# Autodesk Inventor assembly: GP2-100
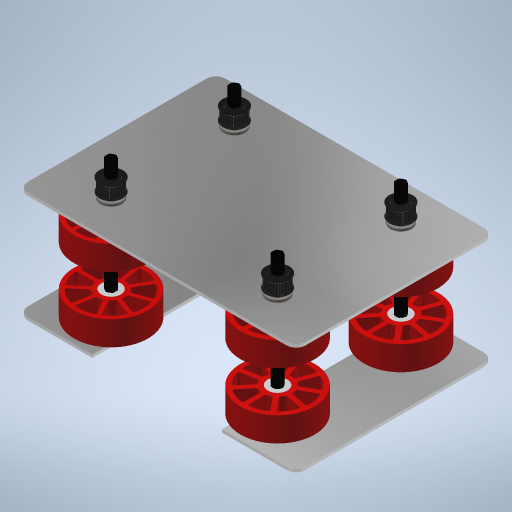
[picture p0: Inventor's stored thumbnail of the model, 512x512]
Saved by Autodesk Inventor 2023.4 (Build 274418000, 418)
## iProperties
Created: 2025-01-12
Part Number: GP2-100
Document SubType Name: Assembly
Designer: jmcintyr
Author: jmcintyr
## Documents named in this file (8)
- C:\Users\jmcintyr\Desktop\2025-ReefScape---CAD\Gripper\GP2\GP2-100.iam
- C:\Users\jmcintyr\Desktop\2025-ReefScape---CAD\Gripper\GP2\GP2-002.ipt
- C:\Users\jmcintyr\Desktop\2025-ReefScape---CAD\Gripper\GP2\GP2-001.ipt
- C:\Users\jmcintyr\Desktop\2025-ReefScape---CAD\COMMON PARTS\BEARINGS\10_25mm_3_8_ThunderHex_ID_x_0_875_OD_x_0_280_WD_Flanged_Bearing_217-5829.ipt
- C:\Users\jmcintyr\Desktop\2025-ReefScape---CAD\Gripper\GP2\GP2-002_MIR4.ipt
- C:\Users\jmcintyr\Desktop\2025-ReefScape---CAD\COMMON PARTS\WHEELS\am-3946 3IN 375Hex Compliant Wheel REV 3.ipt
- C:\Users\jmcintyr\Desktop\2025-ReefScape---CAD\Gripper\GP2\.375_ThunderHex.ipt
- C:\Users\jmcintyr\Desktop\2025-ReefScape---CAD\COMMON PARTS\PULLEYS\gt2\24T_GT2_375_HexBore_9mm_wide_Flanged_Pulley.ipt
## Components (27 placed, 7 different names)
1. GP2-002:1 — Flush:1, Flush:2, Flush:3, Flush:8, Insert:1, Insert:2, Insert:3
2. GP2-001:1 — Flush:8, Insert:1, Insert:4, Insert:5, Insert:8, Insert:9
3. 10_25mm_3_8_ThunderHex_ID_x_0_875_OD_x_0_280_WD_Flanged_Bearing_217-5829:1 — Insert:9, Insert:16, Insert:26
4. 10_25mm_3_8_ThunderHex_ID_x_0_875_OD_x_0_280_WD_Flanged_Bearing_217-5829:2 — Insert:8, Insert:17, Insert:27
5. 10_25mm_3_8_ThunderHex_ID_x_0_875_OD_x_0_280_WD_Flanged_Bearing_217-5829:3 — Insert:5, Insert:14, Insert:25
6. 10_25mm_3_8_ThunderHex_ID_x_0_875_OD_x_0_280_WD_Flanged_Bearing_217-5829:4 — Insert:4, Insert:15, Insert:24
7. 10_25mm_3_8_ThunderHex_ID_x_0_875_OD_x_0_280_WD_Flanged_Bearing_217-5829:5 — Insert:10, Insert:19, Insert:20
8. 10_25mm_3_8_ThunderHex_ID_x_0_875_OD_x_0_280_WD_Flanged_Bearing_217-5829:6 — Insert:11, Insert:18, Insert:23
9. 10_25mm_3_8_ThunderHex_ID_x_0_875_OD_x_0_280_WD_Flanged_Bearing_217-5829:7 — Insert:2, Insert:12, Insert:21
10. 10_25mm_3_8_ThunderHex_ID_x_0_875_OD_x_0_280_WD_Flanged_Bearing_217-5829:8 — Insert:3, Insert:13, Insert:22
11. GP2-002_MIR4:1 — Flush:9, Flush:10, Flush:11, Insert:10, Insert:11
12. am-3946 3IN 375Hex Compliant Wheel REV 3:1 — Insert:15
13. am-3946 3IN 375Hex Compliant Wheel REV 3:2 — Insert:14
14. am-3946 3IN 375Hex Compliant Wheel REV 3:3 — Insert:13
15. am-3946 3IN 375Hex Compliant Wheel REV 3:4 — Insert:12
16. am-3946 3IN 375Hex Compliant Wheel REV 3:5 — Insert:18
17. am-3946 3IN 375Hex Compliant Wheel REV 3:6 — Insert:17
18. am-3946 3IN 375Hex Compliant Wheel REV 3:7 — Insert:16
19. am-3946 3IN 375Hex Compliant Wheel REV 3:8 — Insert:19
20. .375_ThunderHex:1 — Insert:20
21. .375_ThunderHex:2 — Insert:23
22. .375_ThunderHex:3 — Insert:22
23. .375_ThunderHex:4 — Insert:21
24. 24T_GT2_375_HexBore_9mm_wide_Flanged_Pulley:1 — Insert:27
25. 24T_GT2_375_HexBore_9mm_wide_Flanged_Pulley:2 — Insert:24
26. 24T_GT2_375_HexBore_9mm_wide_Flanged_Pulley:3 — Insert:25
27. 24T_GT2_375_HexBore_9mm_wide_Flanged_Pulley:4 — Insert:26
## Relationships (35: Insert 25, Flush 7, Mate 2, Angle 1)
- Mate:1
- Angle:1 (0 deg)
- Flush:1 (-19.05 mm): GP2-002:1
- Mate:2 (85.725 mm)
- Flush:2: GP2-002:1
- Flush:3: GP2-002:1
- Flush:8: GP2-002:1 ↔ GP2-001:1
- Insert:1 (107.95 mm): GP2-002:1 ↔ GP2-001:1
- Insert:2: GP2-002:1 ↔ 10_25mm_3_8_ThunderHex_ID_x_0_875_OD_x_0_280_WD_Flanged_Bearing_217-5829:7
- Insert:3: GP2-002:1 ↔ 10_25mm_3_8_ThunderHex_ID_x_0_875_OD_x_0_280_WD_Flanged_Bearing_217-5829:8
- Insert:4: GP2-001:1 ↔ 10_25mm_3_8_ThunderHex_ID_x_0_875_OD_x_0_280_WD_Flanged_Bearing_217-5829:4
- Insert:5: GP2-001:1 ↔ 10_25mm_3_8_ThunderHex_ID_x_0_875_OD_x_0_280_WD_Flanged_Bearing_217-5829:3
- Insert:8: GP2-001:1 ↔ 10_25mm_3_8_ThunderHex_ID_x_0_875_OD_x_0_280_WD_Flanged_Bearing_217-5829:2
- Insert:9: GP2-001:1 ↔ 10_25mm_3_8_ThunderHex_ID_x_0_875_OD_x_0_280_WD_Flanged_Bearing_217-5829:1
- Flush:9: GP2-002_MIR4:1
- Flush:10: GP2-002_MIR4:1
- Flush:11 (-19.05 mm): GP2-002_MIR4:1
- Insert:10: 10_25mm_3_8_ThunderHex_ID_x_0_875_OD_x_0_280_WD_Flanged_Bearing_217-5829:5 ↔ GP2-002_MIR4:1
- Insert:11: 10_25mm_3_8_ThunderHex_ID_x_0_875_OD_x_0_280_WD_Flanged_Bearing_217-5829:6 ↔ GP2-002_MIR4:1
- Insert:12 (3.175 mm): 10_25mm_3_8_ThunderHex_ID_x_0_875_OD_x_0_280_WD_Flanged_Bearing_217-5829:7 ↔ am-3946 3IN 375Hex Compliant Wheel REV 3:4
- Insert:13 (3.175 mm): 10_25mm_3_8_ThunderHex_ID_x_0_875_OD_x_0_280_WD_Flanged_Bearing_217-5829:8 ↔ am-3946 3IN 375Hex Compliant Wheel REV 3:3
- Insert:14 (9.525 mm): 10_25mm_3_8_ThunderHex_ID_x_0_875_OD_x_0_280_WD_Flanged_Bearing_217-5829:3 ↔ am-3946 3IN 375Hex Compliant Wheel REV 3:2
- Insert:15 (9.525 mm): 10_25mm_3_8_ThunderHex_ID_x_0_875_OD_x_0_280_WD_Flanged_Bearing_217-5829:4 ↔ am-3946 3IN 375Hex Compliant Wheel REV 3:1
- Insert:16 (9.525 mm): 10_25mm_3_8_ThunderHex_ID_x_0_875_OD_x_0_280_WD_Flanged_Bearing_217-5829:1 ↔ am-3946 3IN 375Hex Compliant Wheel REV 3:7
- Insert:17 (9.525 mm): 10_25mm_3_8_ThunderHex_ID_x_0_875_OD_x_0_280_WD_Flanged_Bearing_217-5829:2 ↔ am-3946 3IN 375Hex Compliant Wheel REV 3:6
- Insert:18 (3.175 mm): 10_25mm_3_8_ThunderHex_ID_x_0_875_OD_x_0_280_WD_Flanged_Bearing_217-5829:6 ↔ am-3946 3IN 375Hex Compliant Wheel REV 3:5
- Insert:19 (3.175 mm): 10_25mm_3_8_ThunderHex_ID_x_0_875_OD_x_0_280_WD_Flanged_Bearing_217-5829:5 ↔ am-3946 3IN 375Hex Compliant Wheel REV 3:8
- Insert:20: 10_25mm_3_8_ThunderHex_ID_x_0_875_OD_x_0_280_WD_Flanged_Bearing_217-5829:5 ↔ .375_ThunderHex:1
- Insert:21: 10_25mm_3_8_ThunderHex_ID_x_0_875_OD_x_0_280_WD_Flanged_Bearing_217-5829:7 ↔ .375_ThunderHex:4
- Insert:22: 10_25mm_3_8_ThunderHex_ID_x_0_875_OD_x_0_280_WD_Flanged_Bearing_217-5829:8 ↔ .375_ThunderHex:3
- Insert:23: 10_25mm_3_8_ThunderHex_ID_x_0_875_OD_x_0_280_WD_Flanged_Bearing_217-5829:6 ↔ .375_ThunderHex:2
- Insert:24: 10_25mm_3_8_ThunderHex_ID_x_0_875_OD_x_0_280_WD_Flanged_Bearing_217-5829:4 ↔ 24T_GT2_375_HexBore_9mm_wide_Flanged_Pulley:2
- Insert:25: 10_25mm_3_8_ThunderHex_ID_x_0_875_OD_x_0_280_WD_Flanged_Bearing_217-5829:3 ↔ 24T_GT2_375_HexBore_9mm_wide_Flanged_Pulley:3
- Insert:26: 10_25mm_3_8_ThunderHex_ID_x_0_875_OD_x_0_280_WD_Flanged_Bearing_217-5829:1 ↔ 24T_GT2_375_HexBore_9mm_wide_Flanged_Pulley:4
- Insert:27: 10_25mm_3_8_ThunderHex_ID_x_0_875_OD_x_0_280_WD_Flanged_Bearing_217-5829:2 ↔ 24T_GT2_375_HexBore_9mm_wide_Flanged_Pulley:1
